# Autodesk Inventor assembly: Servo Testing V4
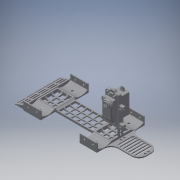
[picture p0: Inventor's stored thumbnail of the model, 180x180]
Saved by Autodesk Inventor 2019 (Build 230136000, 136)
## iProperties
Created: 2018-11-18
Part Number: Servo Testing V4
Document SubType Name: Assembly
Designer: Ashley
Author: Ashley
## Documents named in this file (4)
- C:\Users\Ashley\Desktop\repositories\design\inventor\2018-2019\Tape Measure Braket\Version Four\Servo Testing V4.iam
- C:\Users\Ashley\Desktop\repositories\design\inventor\2018-2019\Tape Measure Braket\Version Five\Bracket Bottom V5.ipt
- C:\Users\Ashley\Desktop\repositories\design\inventor\Imported Components\goBilda\1802SeriesServoFrame.ipt
- C:\Users\Ashley\Desktop\repositories\design\inventor\Imported Components\goBilda\goBildaServo.ipt
## Components (3 placed, 3 different names)
1. Bracket Bottom V5:1
2. 1802SeriesServoFrame:1 — Insert:1, Insert:2
3. goBildaServo:1 — Insert:1, Insert:2
## Relationships (2: Insert 2)
- Insert:1: 1802SeriesServoFrame:1 ↔ goBildaServo:1
- Insert:2: 1802SeriesServoFrame:1 ↔ goBildaServo:1
